# Autodesk Inventor assembly: arm_assembly
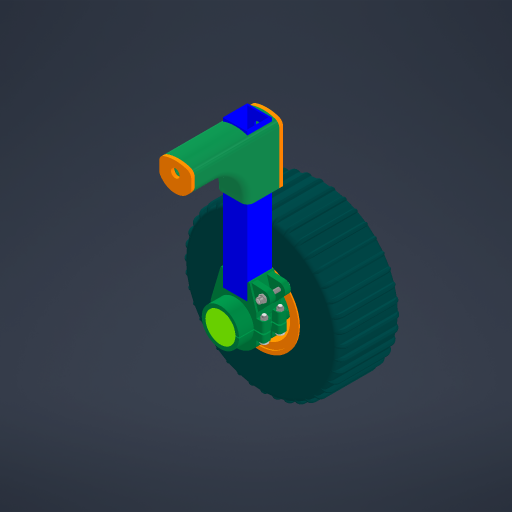
[picture p0: Inventor's stored thumbnail of the model, 512x512]
Saved by Autodesk Inventor 2024 (Build 280153000, 153)
## iProperties
Created: 2023-09-26
Part Number: arm_assembly
Document SubType Name: Assembly
Designer: user
Author: user
## Documents named in this file (5)
- D:\Docs\Robot\3d_v2\machine_body\arm_assembly_r.iam
- D:\Docs\Robot\3d_v2\default_components\motor.ipt
- D:\Docs\Robot\3d_v2\machine_body\arm_assembly\defualt_arm_assembly.iam
- D:\Docs\Robot\3d_v2\machine_body\arm_assembly\wheel_assembly.iam
- D:\Docs\Robot\3d_v2\machine_body\arm_assembly\arm_holder.iam
## Components (4 placed, 4 different names)
1. defualt_arm_assembly:1 [sub-assembly] — Совмещение:1, Совмещение:2, Совмещение:3, Вставка:2, Совмещение:4, Вставка:3
2. wheel_assembly:1 [sub-assembly] — Вставка:1
3. motor:1 — Вставка:1, Вставка:2
4. arm_holder:1 [sub-assembly] — Совмещение:4, Вставка:3
## Relationships (7: Mate 4, Insert 3)
- Совмещение:1 [Mate]: defualt_arm_assembly:1
- Совмещение:2 [Mate]: defualt_arm_assembly:1
- Совмещение:3 [Mate]: defualt_arm_assembly:1
- Вставка:1 [Insert]: wheel_assembly:1 ↔ motor:1
- Вставка:2 [Insert]: defualt_arm_assembly:1 ↔ motor:1
- Совмещение:4 [Mate]: defualt_arm_assembly:1 ↔ arm_holder:1
- Вставка:3 [Insert]: defualt_arm_assembly:1 ↔ arm_holder:1
